# Autodesk Inventor assembly: Matchboxscope_v1
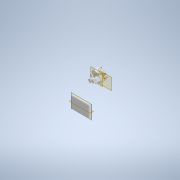
[picture p0: Inventor's stored thumbnail of the model, 180x180]
Saved by Autodesk Inventor 2022 (Build 260153000, 153)
## iProperties
Created: 2022-04-02
Part Number: Matchboxscope_v1
Document SubType Name: Assembly
Designer: Prakash Lab
Author: Prakash Lab
## Documents named in this file (9)
- C:\Users\diederichbenedict\Dropbox\Dokumente\Promotion\PROJECTS\Matchboxscope\INVENTOR\Matchboxscope_v1.iam
- C:\Users\diederichbenedict\Dropbox\Dokumente\Promotion\PROJECTS\Matchboxscope\INVENTOR\Matchboxscope_middle2_v1.ipt
- C:\Users\diederichbenedict\Dropbox\Dokumente\Promotion\PROJECTS\Matchboxscope\INVENTOR\Matchboxscope_Lightperiscope_V0.ipt
- C:\Users\diederichbenedict\Dropbox\Dokumente\Promotion\PROJECTS\Matchboxscope\INVENTOR\Matchboxscope_Lightperiscope_long_V0.ipt
- C:\Users\diederichbenedict\Dropbox\Dokumente\Promotion\PROJECTS\Matchboxscope\INVENTOR\Matchboxscope_bottom_v0.ipt
- C:\Users\diederichbenedict\Dropbox\Dokumente\Promotion\PROJECTS\Matchboxscope\INVENTOR\00_ESP3-CAM.iam
- C:\Users\diederichbenedict\Dropbox\Dokumente\Promotion\PROJECTS\Matchboxscope\INVENTOR\Matchboxscope_sample_v1.ipt
- C:\Users\diederichbenedict\Dropbox\Dokumente\Promotion\PROJECTS\Matchboxscope\INVENTOR\Matchboxscope_lenstube_v0.ipt
- C:\Users\diederichbenedict\Dropbox\Dokumente\Promotion\PROJECTS\Matchboxscope\INVENTOR\00_Powerbank.ipt
## Components (8 placed, 8 different names)
1. Matchboxscope_middle2_v1:1 — Insert:1, Angle:1, Mate:5, Flush:2, Flush:3
2. Matchboxscope_Lightperiscope_V0:1
3. Matchboxscope_Lightperiscope_long_V0:1 — Insert:2, Angle:2
4. Matchboxscope_bottom_v0:1 — Mate:1, Mate:2, Mate:3, Mate:4, Flush:1, Mate:5
5. 00_ESP3-CAM:1 [sub-assembly] — Mate:4, Flush:1, Insert:1
6. Matchboxscope_sample_v1:1 — Flush:2, Flush:3, Insert:2, Angle:2, Mate:6
7. Matchboxscope_lenstube_v0:1 — Mate:6
8. 00_Powerbank:1
## Relationships (13: Mate 6, Flush 3, Insert 2, Angle 2)
- Mate:1: Matchboxscope_bottom_v0:1
- Mate:2: Matchboxscope_bottom_v0:1
- Mate:3: Matchboxscope_bottom_v0:1
- Mate:4: Matchboxscope_bottom_v0:1 ↔ 00_ESP3-CAM:1
- Flush:1: Matchboxscope_bottom_v0:1 ↔ 00_ESP3-CAM:1
- Insert:1: Matchboxscope_middle2_v1:1 ↔ 00_ESP3-CAM:1
- Angle:1 (0 deg): Matchboxscope_middle2_v1:1
- Mate:5: Matchboxscope_middle2_v1:1 ↔ Matchboxscope_bottom_v0:1
- Flush:2: Matchboxscope_middle2_v1:1 ↔ Matchboxscope_sample_v1:1
- Flush:3: Matchboxscope_middle2_v1:1 ↔ Matchboxscope_sample_v1:1
- Insert:2 (-3 mm): Matchboxscope_Lightperiscope_long_V0:1 ↔ Matchboxscope_sample_v1:1
- Angle:2 (90 deg): Matchboxscope_Lightperiscope_long_V0:1 ↔ Matchboxscope_sample_v1:1
- Mate:6: Matchboxscope_sample_v1:1 ↔ Matchboxscope_lenstube_v0:1
